# Autodesk Inventor assembly: 初段_多段ギア
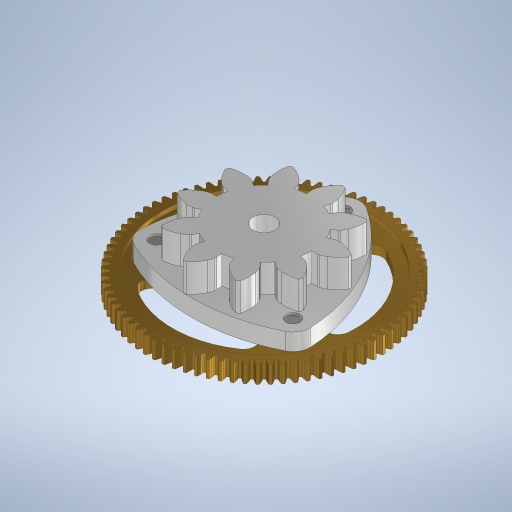
[picture p0: Inventor's stored thumbnail of the model, 512x512]
Saved by Autodesk Inventor 2023 (Build 270158030, 158C)
## iProperties
Created: 2022-01-11
Part Number: 初段_多段ギア
Document SubType Name: Assembly
Designer: acps
Mass: 20.0582 g
Surface Area: 47.1647 cm^2
Volume: 4.94221 cm^3
Density: 4.05855 g/cm^3
Author: acps
## Documents named in this file (4)
- C:\Users\muzho\Documents\srdc\srdc_2\脚\ギア\初段_多段ギア.iam
- C:\Users\muzho\Documents\srdc\srdc_2\脚\ギア\多段ギアm2z10t8.ipt
- C:\Users\muzho\Documents\srdc\srdc_2\脚\ギア\初段ギアm0.5z80.ipt
- C:\Users\muzho\Documents\srdc\srdc_2\ねじ\M3L4　超極低頭.ipt
## Components (5 placed, 3 different names)
1. 多段ギアm2z10t8:1 — Mate:1, Mate:2, Insert:1, メイト:3
2. 初段ギアm0.5z80:1 — Mate:1, Mate:2, Insert:1, メイト:3, 挿入:2, 挿入:3, 挿入:4
3. M3L4　超極低頭:1 — 挿入:4
4. M3L4　超極低頭:2 — 挿入:3
5. M3L4　超極低頭:3 — 挿入:2
## Relationships (7: Insert 4, Mate 3)
- Mate:1: 多段ギアm2z10t8:1 ↔ 初段ギアm0.5z80:1
- Mate:2: 多段ギアm2z10t8:1 ↔ 初段ギアm0.5z80:1
- Insert:1: 多段ギアm2z10t8:1 ↔ 初段ギアm0.5z80:1
- メイト:3 [Mate]: 多段ギアm2z10t8:1 ↔ 初段ギアm0.5z80:1
- 挿入:2 [Insert]: 初段ギアm0.5z80:1 ↔ M3L4　超極低頭:3
- 挿入:3 [Insert]: 初段ギアm0.5z80:1 ↔ M3L4　超極低頭:2
- 挿入:4 [Insert]: 初段ギアm0.5z80:1 ↔ M3L4　超極低頭:1
